# Autodesk Inventor assembly: EDMPumpRegionAssembly
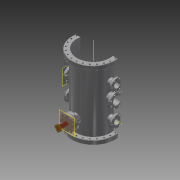
[picture p0: Inventor's stored thumbnail of the model, 180x180]
Saved by Autodesk Inventor 2015 SP1 (Build 190203100, 203)
## iProperties
Created: 2014-03-24
Part Number: EDMPumpRegionAssembly
Document SubType Name: Assembly
Designer: jad211
Author: jad211
## Documents named in this file (8)
- C:\ColdMatter\CADFiles\EDM Machine\Pumping Region\Pumping Region\EDMPumpRegionAssembly.iam
- C:\ColdMatter\CADFiles\EDM Machine\Pumping Region\Pumping Region\NewHorn.ipt
- C:\ColdMatter\CADFiles\EDM Machine\Pumping Region\Pumping Region\WG18FLANGECutDown.ipt
- C:\ColdMatter\CADFiles\EDM Machine\Beamline\Chamber parts\hudson chamber actual size.ipt
- C:\ColdMatter\CADFiles\EDM Machine\Pumping Region\Pumping Region\FlangedWaveguide.iam
- C:\ColdMatter\CADFiles\EDM Machine\Pumping Region\Pumping Region\3-38sWithWG18Hole.ipt
- C:\ColdMatter\CADFiles\EDM Machine\Pumping Region\rfCoilSmaller.ipt
- C:\ColdMatter\CADFiles\EDM Machine\Pumping Region\rfCoil.ipt
## Components (9 placed, 7 different names)
1. hudson chamber actual size:1 — Mate:12, Flush:15, Angle:1, Mate:13, Mate:24, Mate:27, Mate:29, Mate:30, Mate:31, Mate:33, Mate:35, Mate:36, Mate:39
2. NewHorn:1 — Mate:14, Angle:2, Flush:17, Mate:17, Mate:18, Mate:19, Mate:21, Flush:20
3. WG18FLANGECutDown:1 — Flush:17, Mate:18, Mate:19, Mate:20
4. FlangedWaveguide:2 [sub-assembly] — Mate:17, Mate:20, Mate:21, Mate:22, Mate:23
5. 3-38sWithWG18Hole:1 — Mate:22, Mate:23, Mate:24
6. rfCoilSmaller:1 — Mate:25, Mate:26, Mate:28, Mate:30
7. rfCoilSmaller:2 — Mate:29, Mate:32, Mate:33
8. rfCoil:1 — Mate:34, Mate:35, Mate:36
9. rfCoil:2 — Mate:37, Mate:38, Mate:39
## Relationships (35: Mate 26, Flush 5, Angle 4)
- Flush:8 (3 mm)
- Mate:12: hudson chamber actual size:1
- Flush:15: hudson chamber actual size:1
- Flush:16 (-304.8 mm)
- Angle:1 (0 deg): hudson chamber actual size:1
- Mate:13: hudson chamber actual size:1
- Mate:14: NewHorn:1
- Angle:2 (0 deg): NewHorn:1
- Flush:17: NewHorn:1 ↔ WG18FLANGECutDown:1
- Mate:17: NewHorn:1 ↔ FlangedWaveguide:2
- Mate:18: NewHorn:1 ↔ WG18FLANGECutDown:1
- Mate:19: NewHorn:1 ↔ WG18FLANGECutDown:1
- Mate:20: WG18FLANGECutDown:1 ↔ FlangedWaveguide:2
- Mate:21: NewHorn:1 ↔ FlangedWaveguide:2
- Flush:20 (-25 mm): NewHorn:1
- Mate:22: FlangedWaveguide:2 ↔ 3-38sWithWG18Hole:1
- Mate:23: FlangedWaveguide:2 ↔ 3-38sWithWG18Hole:1
- Mate:24: hudson chamber actual size:1 ↔ 3-38sWithWG18Hole:1
- Mate:25: rfCoilSmaller:1
- Mate:26: rfCoilSmaller:1
- Mate:27: hudson chamber actual size:1
- Angle:3 (45 deg)
- Mate:28: rfCoilSmaller:1
- Mate:29: hudson chamber actual size:1 ↔ rfCoilSmaller:2
- Mate:30: hudson chamber actual size:1 ↔ rfCoilSmaller:1
- Mate:31: hudson chamber actual size:1
- Angle:4 (90 deg)
- Mate:32: rfCoilSmaller:2
- Mate:33: hudson chamber actual size:1 ↔ rfCoilSmaller:2
- Mate:34: rfCoil:1
- Mate:35: hudson chamber actual size:1 ↔ rfCoil:1
- Mate:36: hudson chamber actual size:1 ↔ rfCoil:1
- Mate:37: rfCoil:2
- Mate:38: rfCoil:2
- Mate:39: hudson chamber actual size:1 ↔ rfCoil:2
